# Autodesk Inventor assembly: carrier12
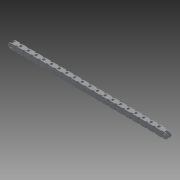
[picture p0: Inventor's stored thumbnail of the model, 180x180]
Saved by Autodesk Inventor 2013 (Build 170138000, 138)
## iProperties
Created: 2013-01-14
Part Number: carrier12
Document SubType Name: Assembly
Designer: Istvan
Author: Istvan
## Documents named in this file (2)
- C:\Users\istvan.burbank\Documents\GitHub\Crown-Fire\CAD\Electronics\carrier\carrier12.iam
- C:\Users\istvan.burbank\Documents\GitHub\Crown-Fire\CAD\Electronics\carrier\carrierSegment.ipt
## Components (20 placed, 1 different names)
1. carrierSegment:1 — Mate:1, Mate:17
2. carrierSegment:2 — Mate:1, Mate:2, Mate:17, Mate:18
3. carrierSegment:3 — Mate:2, Mate:3, Mate:18, Mate:19
4. carrierSegment:4 — Mate:3, Mate:4, Mate:19, Mate:20
5. carrierSegment:5 — Mate:4, Mate:5, Mate:20, Mate:21
6. carrierSegment:6 — Mate:5, Mate:6, Mate:21, Mate:22
7. carrierSegment:7 — Mate:6, Mate:7, Mate:22, Mate:23
8. carrierSegment:8 — Mate:7, Mate:8, Mate:23, Mate:24
9. carrierSegment:9 — Mate:8, Mate:9, Mate:24, Mate:25
10. carrierSegment:10 — Mate:9, Mate:10, Mate:25, Mate:26
11. carrierSegment:11 — Mate:10, Mate:11, Mate:26, Mate:27
12. carrierSegment:12 — Mate:11, Mate:12, Mate:27, Mate:28
13. carrierSegment:13 — Mate:12, Mate:13, Mate:28, Mate:29
14. carrierSegment:14 — Mate:13, Mate:14, Mate:29, Mate:30
15. carrierSegment:15 — Mate:14, Mate:30, Mate:31, Mate:37
16. carrierSegment:16 — Mate:31, Mate:32, Mate:37, Mate:38
17. carrierSegment:17 — Mate:32, Mate:33, Mate:38, Mate:39
18. carrierSegment:18 — Mate:33, Mate:34, Mate:39, Mate:40
19. carrierSegment:19 — Mate:34, Mate:35, Mate:40, Mate:41
20. carrierSegment:20 — Mate:35, Mate:41
## Relationships (38: Mate 38)
- Mate:1: carrierSegment:1 ↔ carrierSegment:2
- Mate:2: carrierSegment:2 ↔ carrierSegment:3
- Mate:3: carrierSegment:3 ↔ carrierSegment:4
- Mate:4: carrierSegment:4 ↔ carrierSegment:5
- Mate:5: carrierSegment:5 ↔ carrierSegment:6
- Mate:6: carrierSegment:6 ↔ carrierSegment:7
- Mate:7: carrierSegment:7 ↔ carrierSegment:8
- Mate:8: carrierSegment:8 ↔ carrierSegment:9
- Mate:9: carrierSegment:9 ↔ carrierSegment:10
- Mate:10: carrierSegment:10 ↔ carrierSegment:11
- Mate:11: carrierSegment:11 ↔ carrierSegment:12
- Mate:12: carrierSegment:12 ↔ carrierSegment:13
- Mate:13: carrierSegment:13 ↔ carrierSegment:14
- Mate:14: carrierSegment:14 ↔ carrierSegment:15
- Mate:17: carrierSegment:1 ↔ carrierSegment:2
- Mate:18: carrierSegment:2 ↔ carrierSegment:3
- Mate:19: carrierSegment:3 ↔ carrierSegment:4
- Mate:20: carrierSegment:4 ↔ carrierSegment:5
- Mate:21: carrierSegment:5 ↔ carrierSegment:6
- Mate:22: carrierSegment:6 ↔ carrierSegment:7
- Mate:23: carrierSegment:7 ↔ carrierSegment:8
- Mate:24: carrierSegment:8 ↔ carrierSegment:9
- Mate:25: carrierSegment:9 ↔ carrierSegment:10
- Mate:26: carrierSegment:10 ↔ carrierSegment:11
- Mate:27: carrierSegment:11 ↔ carrierSegment:12
- Mate:28: carrierSegment:12 ↔ carrierSegment:13
- Mate:29: carrierSegment:13 ↔ carrierSegment:14
- Mate:30: carrierSegment:14 ↔ carrierSegment:15
- Mate:31: carrierSegment:15 ↔ carrierSegment:16
- Mate:32: carrierSegment:16 ↔ carrierSegment:17
- Mate:33: carrierSegment:17 ↔ carrierSegment:18
- Mate:34: carrierSegment:18 ↔ carrierSegment:19
- Mate:35: carrierSegment:19 ↔ carrierSegment:20
- Mate:37: carrierSegment:15 ↔ carrierSegment:16
- Mate:38: carrierSegment:16 ↔ carrierSegment:17
- Mate:39: carrierSegment:17 ↔ carrierSegment:18
- Mate:40: carrierSegment:18 ↔ carrierSegment:19
- Mate:41: carrierSegment:19 ↔ carrierSegment:20
